# Autodesk Inventor assembly: Z-axis Drive Assembly
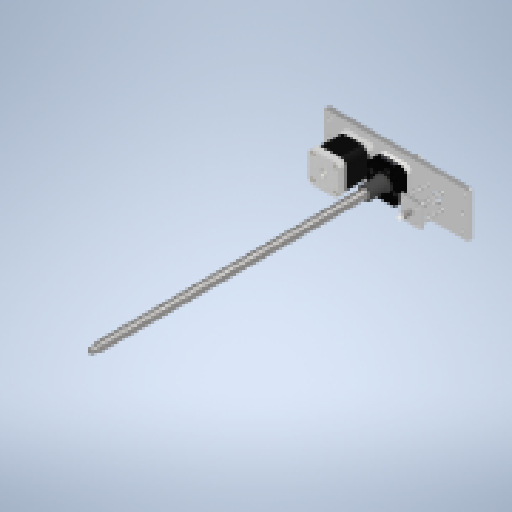
[picture p0: Inventor's stored thumbnail of the model, 512x512]
Saved by Autodesk Inventor 2024 (Build 280153000, 153)
## iProperties
Created: 2024-12-31
Part Number: Z-axis Drive Assembly
Document SubType Name: Assembly
Designer: Ishaan
Author: Ishaan
## Documents named in this file (12)
- E:\Projects\Axiom--IDEX-3D-Printer\CAD\02 - Z-axis\Z-axis Drive Assembly.iam
- E:\Projects\Axiom--IDEX-3D-Printer\CAD\02 - Z-axis\Z-Axis Drive Mount RevII.ipt
- E:\Projects\Axiom--IDEX-3D-Printer\CAD\00 - COTS Components\FK10\FK10-C5\FK10-C5\FK10-C5.iam
- E:\Projects\Axiom--IDEX-3D-Printer\CAD\00 - COTS Components\SFU1204 Ballscrew\1204 Ballscrew.ipt
- E:\Projects\Axiom--IDEX-3D-Printer\CAD\00 - COTS Components\6mm 40T GT2 Timing Pulley SFU1204 Bore\6mm 40T GT2 Timing Pulley SFU1204 Bore.ipt
- E:\Projects\Axiom--IDEX-3D-Printer\CAD\02 - Z-axis\Ballscrew Spacer.ipt
- E:\Projects\Axiom--IDEX-3D-Printer\CAD\00 - COTS Components\6mm 20T GT2 Timing Pulley 5mm Bore\6mm 20T GT2 Timing Pulley 5mm Bore.ipt
- E:\Projects\Axiom--IDEX-3D-Printer\CAD\00 - COTS Components\NEMA 17 - Long\NEMA 17 Long.ipt
- E:\Projects\Axiom--IDEX-3D-Printer\CAD\00 - COTS Components\Hardware\M3 30mm Standoff.ipt
- E:\Projects\Axiom--IDEX-3D-Printer\CAD\02 - Z-axis\Inductive Sensor Plate.ipt
- E:\Projects\Axiom--IDEX-3D-Printer\CAD\02 - Z-axis\Z-screw Bump Stop.ipt
- E:\Projects\Axiom--IDEX-3D-Printer\CAD\00 - COTS Components\6mm Inductive Probe\6mm Inductive Probe.ipt
## Components (14 placed, 11 different names)
1. Z-Axis Drive Mount RevII:1 — Insert:9, Insert:10, Insert:11, Insert:12, Insert:13, Insert:14, Flush:2
2. NEMA 17 Long:1
3. FK10-C5:1 [sub-assembly] — Insert:3, Insert:4, Insert:7, Insert:8, Insert:17
4. 1204 Ballscrew:1 — Insert:3
5. 6mm 40T GT2 Timing Pulley SFU1204 Bore:1 — Insert:4, Flush:1
6. Ballscrew Spacer:1 — Insert:7, Insert:8, Insert:9, Insert:10
7. 6mm 20T GT2 Timing Pulley 5mm Bore:1 — Flush:1
8. M3 30mm Standoff:1 — Insert:11, Insert:15
9. M3 30mm Standoff:2 — Insert:12
10. M3 30mm Standoff:3 — Insert:13, Insert:16
11. M3 30mm Standoff:4 — Insert:14
12. Inductive Sensor Plate:1 — Insert:15, Insert:16, Mate:2
13. Z-screw Bump Stop:1 — Insert:17
14. 6mm Inductive Probe:1 — Mate:2, Flush:2
## Relationships (19: Insert 15, Mate 2, Flush 2)
- Insert:3: FK10-C5:1 ↔ 1204 Ballscrew:1
- Insert:4: FK10-C5:1 ↔ 6mm 40T GT2 Timing Pulley SFU1204 Bore:1
- [Insert]: Z-Axis Drive Mount RevII:1 ↔ NEMA 17 Long:1
- [Insert]: Z-Axis Drive Mount RevII:1 ↔ NEMA 17 Long:1
- Insert:7: FK10-C5:1 ↔ Ballscrew Spacer:1
- Insert:8: FK10-C5:1 ↔ Ballscrew Spacer:1
- [Mate]: NEMA 17 Long:1 ↔ 6mm 20T GT2 Timing Pulley 5mm Bore:1
- Flush:1: 6mm 40T GT2 Timing Pulley SFU1204 Bore:1 ↔ 6mm 20T GT2 Timing Pulley 5mm Bore:1
- Insert:9: Z-Axis Drive Mount RevII:1 ↔ Ballscrew Spacer:1
- Insert:10: Z-Axis Drive Mount RevII:1 ↔ Ballscrew Spacer:1
- Insert:11: Z-Axis Drive Mount RevII:1 ↔ M3 30mm Standoff:1
- Insert:12: Z-Axis Drive Mount RevII:1 ↔ M3 30mm Standoff:2
- Insert:13: Z-Axis Drive Mount RevII:1 ↔ M3 30mm Standoff:3
- Insert:14: Z-Axis Drive Mount RevII:1 ↔ M3 30mm Standoff:4
- Insert:15: M3 30mm Standoff:1 ↔ Inductive Sensor Plate:1
- Insert:16: M3 30mm Standoff:3 ↔ Inductive Sensor Plate:1
- Insert:17: FK10-C5:1 ↔ Z-screw Bump Stop:1
- Mate:2: Inductive Sensor Plate:1 ↔ 6mm Inductive Probe:1
- Flush:2 (-49 mm): Z-Axis Drive Mount RevII:1 ↔ 6mm Inductive Probe:1
